# Autodesk Inventor assembly: Table
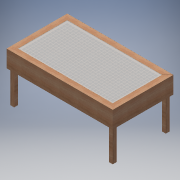
[picture p0: Inventor's stored thumbnail of the model, 180x180]
Saved by Autodesk Inventor 2016 (Build 200138000, 138)
## iProperties
Created: 2016-02-08
Part Number: Table
Document SubType Name: Assembly
Designer: ron
Author: ron
## Documents named in this file (16)
- C:\Users\ron\Desktop\Table\Table.iam
- C:\Users\ron\Desktop\Table\Parts\LedBoard.ipt
- C:\Users\ron\Desktop\Table\Parts\DividerWidth.ipt
- C:\Users\ron\Desktop\Table\Parts\DividerLength.ipt
- C:\Users\ron\Desktop\Table\Parts\Acrylitep95.ipt
- C:\Users\ron\Desktop\Table\Parts\LegStandard.ipt
- C:\Users\ron\Desktop\Table\Parts\Glass.ipt
- C:\Users\ron\Desktop\Table\Parts\LegOutlet.ipt
- C:\Users\ron\Desktop\Table\Parts\SideWidth.ipt
- C:\Users\ron\Desktop\Table\Parts\SideLength.ipt
- C:\Users\ron\Desktop\Table\Parts\SideWidthOutlet.ipt
- C:\Users\ron\Desktop\Table\Parts\SideLengthOutlet.ipt
- C:\Users\ron\Desktop\Table\Parts\SupportWedge.ipt
- C:\Users\ron\Desktop\Table\Parts\Bottom.ipt
- C:\Users\ron\Desktop\Table\Parts\PowerSupply.ipt
- C:\Users\ron\Desktop\Table\Parts\Magnet.ipt
## Components (72 placed, 15 different names)
1. LedBoard:1 — Flush:1, Flush:2, Flush:3, Flush:4, Flush:5, Flush:7, Flush:8, Flush:10, Flush:11, Flush:13, Flush:14, Flush:16, Flush:17, Flush:19, Flush:20, Flush:22, Flush:23, Flush:25, Flush:26, Flush:28, Flush:29, Flush:31, Flush:32, Flush:34, Flush:36, Flush:37, Flush:38, Flush:40, Flush:41, Flush:43, Flush:44, Flush:46, Flush:47, Flush:49, Flush:50, Flush:52, Flush:53, Flush:55, Flush:56, Flush:58, Flush:59, Flush:61, Flush:62, Flush:64, Flush:65, Flush:67, Flush:68, Flush:70, Flush:71, Flush:73, Flush:74, Flush:76, Flush:77, Flush:79, Flush:80, Flush:82, Flush:83, Flush:85, Flush:86, Flush:88, Flush:89, Flush:91, Flush:92, Flush:94, Flush:96, Mate:1, Flush:97, Flush:98, Mate:2, Flush:99, Mate:3, Flush:101, Mate:4, Flush:103, Mate:5, Flush:105, Mate:6, Flush:107, Flush:109, Mate:7, Mate:8, Flush:111, Mate:9, Flush:113, Mate:10, Flush:115, Mate:11, Flush:117, Mate:12, Flush:119, Mate:13, Flush:121, Mate:14, Flush:123, Mate:15, Flush:125, Flush:127, Flush:128, Mate:17, Mate:18, Mate:22, Mate:23, Mate:25, Mate:26, Mate:30, Mate:60, Mate:61, Mate:64, Mate:70, Mate:73, Mate:76, Mate:79
2. DividerWidth:1 — Flush:64, Flush:65, Flush:66, Flush:69
3. DividerWidth:2 — Flush:58, Flush:59, Flush:60, Flush:63
4. DividerWidth:3 — Flush:40, Flush:41, Flush:42, Flush:45
5. DividerWidth:4 — Flush:31, Flush:32, Flush:33, Flush:35
6. DividerWidth:5 — Flush:70, Flush:71, Flush:72, Flush:75
7. DividerWidth:6 — Flush:61, Flush:62, Flush:63, Flush:66
8. DividerWidth:7 — Flush:49, Flush:50, Flush:51, Flush:54
9. DividerWidth:8 — Flush:19, Flush:20, Flush:21, Flush:24
10. DividerWidth:9 — Flush:28, Flush:29, Flush:30, Flush:33
11. DividerWidth:10 — Flush:34, Flush:35, Flush:36, Flush:39, Mate:16
12. DividerWidth:11 — Flush:73, Flush:74, Flush:75, Flush:78
13. DividerWidth:12 — Flush:79, Flush:80, Flush:81, Flush:84
14. DividerWidth:13 — Flush:85, Flush:86, Flush:87, Flush:90
15. DividerWidth:14 — Flush:52, Flush:53, Flush:54, Flush:57
16. DividerWidth:15 — Flush:46, Flush:47, Flush:48, Flush:51
17. DividerWidth:16 — Flush:10, Flush:11, Flush:12, Flush:15
18. DividerWidth:17 — Flush:7, Flush:8, Flush:9, Flush:12
19. DividerWidth:18 — Flush:13, Flush:14, Flush:15, Flush:18, Flush:21
20. DividerWidth:19 — Flush:1, Flush:2, Flush:3, Flush:6
21. DividerWidth:20 — Flush:43, Flush:44, Flush:45, Flush:48
22. DividerWidth:21 — Flush:55, Flush:56, Flush:57, Flush:60
23. DividerWidth:22 — Flush:25, Flush:26, Flush:27, Flush:30
24. DividerWidth:23 — Flush:4, Flush:5, Flush:6, Flush:9
25. DividerWidth:24 — Flush:16, Flush:17, Flush:18
26. DividerWidth:25 — Flush:22, Flush:23, Flush:24, Flush:27
27. DividerWidth:26 — Flush:37, Flush:38, Flush:39, Flush:42
28. DividerWidth:27 — Flush:67, Flush:68, Flush:69, Flush:72
29. DividerWidth:28 — Flush:76, Flush:77, Flush:78, Flush:81
30. DividerWidth:29 — Flush:82, Flush:83, Flush:84, Flush:87
31. DividerWidth:30 — Flush:91, Flush:92, Flush:93, Flush:95
32. DividerWidth:31 — Flush:88, Flush:89, Flush:90, Flush:93
33. DividerLength:1 — Mate:5, Flush:105, Flush:106, Flush:108
34. DividerLength:2 — Mate:10, Flush:115, Flush:116, Flush:118
35. DividerLength:3 — Mate:1, Flush:97, Flush:98, Flush:100
36. DividerLength:4 — Mate:11, Flush:117, Flush:118, Flush:120
37. DividerLength:5 — Flush:109, Mate:7, Flush:110, Flush:112
38. DividerLength:6 — Mate:3, Flush:101, Flush:102, Flush:104
39. DividerLength:7 — Mate:13, Flush:121, Flush:122, Flush:124
40. DividerLength:8 — Mate:8, Flush:111, Flush:112, Flush:114
41. DividerLength:9 — Mate:4, Flush:103, Flush:104, Flush:106
42. DividerLength:10 — Mate:12, Flush:119, Flush:120, Flush:122
43. DividerLength:11 — Mate:15, Flush:125, Flush:126
44. DividerLength:12 — Mate:14, Flush:123, Flush:124, Flush:126
45. DividerLength:13 — Mate:9, Flush:113, Flush:114, Flush:116
46. DividerLength:14 — Mate:2, Flush:99, Flush:100, Flush:102
47. DividerLength:15 — Mate:6, Flush:107, Flush:108, Flush:110
48. DividerWidth:32 — Flush:94, Flush:95, Flush:96
49. Acrylitep95:1 — Flush:127, Mate:16, Flush:128, Mate:19, Mate:20, Flush:129, Flush:130, Mate:21, Mate:24, Mate:31, Mate:39, Mate:59, Mate:62, Mate:68
50. LegStandard:1 — Mate:21, Mate:22, Mate:23, Mate:89, Mate:90, Flush:136
51. LegStandard:2 — Mate:24, Mate:25, Mate:26, Mate:91, Mate:92, Flush:137
52. LegStandard:3 — Mate:17, Mate:18, Mate:19, Mate:85, Mate:86, Flush:134
53. Glass:1 — Mate:20, Flush:129, Flush:130, Mate:32, Mate:41, Mate:42, Mate:65
54. SideWidth:1 — Mate:30, Mate:31, Mate:32, Mate:42, Mate:66, Mate:69, Mate:77, Mate:80, Mate:97, Mate:98, Mate:99
55. SideLength:2 — Mate:39, Mate:41, Mate:63, Mate:66, Mate:75, Mate:78, Mate:84, Mate:93, Mate:94, Flush:138, Mate:100, Mate:101, Mate:102
56. LegOutlet:1 — Mate:59, Mate:60, Mate:61, Mate:87, Mate:88, Flush:135
57. SideWidthOutlet:1 — Mate:62, Mate:63, Mate:64, Mate:65, Mate:67, Mate:71, Mate:74, Flush:133, Mate:83, Mate:95, Flush:139, Mate:96
58. SideLengthOutlet:1 — Mate:67, Mate:68, Mate:69, Mate:72, Mate:81
59. SupportWedge:1 — Mate:76, Mate:77, Mate:78
60. SupportWedge:2 — Mate:73, Mate:74, Mate:75
61. SupportWedge:3 — Mate:79, Mate:80, Mate:81
62. SupportWedge:4 — Mate:70, Mate:71, Mate:72
63. Bottom:1 — Mate:82, Flush:131, Flush:132, Flush:133, Mate:83, Mate:84
64. PowerSupply:1 — Mate:82, Flush:131, Flush:132
65. Magnet:1 — Mate:93, Mate:94, Flush:138
66. Magnet:2 — Mate:95, Flush:139, Mate:96
67. Magnet:3 — Mate:85, Mate:86, Flush:134
68. Magnet:4 — Mate:89, Mate:90, Flush:136
69. Magnet:5 — Mate:87, Mate:88, Flush:135
70. Magnet:6 — Mate:91, Mate:92, Flush:137
71. Magnet:7 — Mate:97, Mate:98, Mate:99
72. Magnet:8 — Mate:100, Mate:101, Mate:102
## Relationships (215: Flush 139, Mate 76)
- Flush:1 (-50.8 mm): LedBoard:1 ↔ DividerWidth:19
- Flush:2: LedBoard:1 ↔ DividerWidth:19
- Flush:3 (34.925 mm): LedBoard:1 ↔ DividerWidth:19
- Flush:4: LedBoard:1 ↔ DividerWidth:23
- Flush:5 (-50.8 mm): LedBoard:1 ↔ DividerWidth:23
- Flush:6 (38.1 mm): DividerWidth:19 ↔ DividerWidth:23
- Flush:7 (-50.8 mm): LedBoard:1 ↔ DividerWidth:17
- Flush:8: LedBoard:1 ↔ DividerWidth:17
- Flush:9 (38.1 mm): DividerWidth:17 ↔ DividerWidth:23
- Flush:10 (-50.8 mm): LedBoard:1 ↔ DividerWidth:16
- Flush:11: LedBoard:1 ↔ DividerWidth:16
- Flush:12 (38.1 mm): DividerWidth:16 ↔ DividerWidth:17
- Flush:13 (-50.8 mm): LedBoard:1 ↔ DividerWidth:18
- Flush:14: LedBoard:1 ↔ DividerWidth:18
- Flush:15 (38.1 mm): DividerWidth:16 ↔ DividerWidth:18
- Flush:16 (-50.8 mm): LedBoard:1 ↔ DividerWidth:24
- Flush:17: LedBoard:1 ↔ DividerWidth:24
- Flush:18 (-38.1 mm): DividerWidth:18 ↔ DividerWidth:24
- Flush:19 (-50.8 mm): LedBoard:1 ↔ DividerWidth:8
- Flush:20: LedBoard:1 ↔ DividerWidth:8
- Flush:21 (38.1 mm): DividerWidth:8 ↔ DividerWidth:18
- Flush:22 (-50.8 mm): LedBoard:1 ↔ DividerWidth:25
- Flush:23: LedBoard:1 ↔ DividerWidth:25
- Flush:24 (38.1 mm): DividerWidth:8 ↔ DividerWidth:25
- Flush:25 (-50.8 mm): LedBoard:1 ↔ DividerWidth:22
- Flush:26: LedBoard:1 ↔ DividerWidth:22
- Flush:27 (38.1 mm): DividerWidth:22 ↔ DividerWidth:25
- Flush:28 (-50.8 mm): LedBoard:1 ↔ DividerWidth:9
- Flush:29: LedBoard:1 ↔ DividerWidth:9
- Flush:30 (38.1 mm): DividerWidth:9 ↔ DividerWidth:22
- Flush:31 (-50.8 mm): LedBoard:1 ↔ DividerWidth:4
- Flush:32: LedBoard:1 ↔ DividerWidth:4
- Flush:33 (38.1 mm): DividerWidth:4 ↔ DividerWidth:9
- Flush:34: LedBoard:1 ↔ DividerWidth:10
- Flush:35 (38.1 mm): DividerWidth:4 ↔ DividerWidth:10
- Flush:36 (-50.8 mm): LedBoard:1 ↔ DividerWidth:10
- Flush:37: LedBoard:1 ↔ DividerWidth:26
- Flush:38 (-50.8 mm): LedBoard:1 ↔ DividerWidth:26
- Flush:39 (38.1 mm): DividerWidth:10 ↔ DividerWidth:26
- Flush:40: LedBoard:1 ↔ DividerWidth:3
- Flush:41 (-50.8 mm): LedBoard:1 ↔ DividerWidth:3
- Flush:42 (38.1 mm): DividerWidth:3 ↔ DividerWidth:26
- Flush:43: LedBoard:1 ↔ DividerWidth:20
- Flush:44 (-50.8 mm): LedBoard:1 ↔ DividerWidth:20
- Flush:45 (38.1 mm): DividerWidth:3 ↔ DividerWidth:20
- Flush:46: LedBoard:1 ↔ DividerWidth:15
- Flush:47 (-50.8 mm): LedBoard:1 ↔ DividerWidth:15
- Flush:48 (38.1 mm): DividerWidth:15 ↔ DividerWidth:20
- Flush:49: LedBoard:1 ↔ DividerWidth:7
- Flush:50 (-50.8 mm): LedBoard:1 ↔ DividerWidth:7
- Flush:51 (38.1 mm): DividerWidth:7 ↔ DividerWidth:15
- Flush:52: LedBoard:1 ↔ DividerWidth:14
- Flush:53 (-50.8 mm): LedBoard:1 ↔ DividerWidth:14
- Flush:54 (38.1 mm): DividerWidth:7 ↔ DividerWidth:14
- Flush:55: LedBoard:1 ↔ DividerWidth:21
- Flush:56 (-50.8 mm): LedBoard:1 ↔ DividerWidth:21
- Flush:57 (38.1 mm): DividerWidth:14 ↔ DividerWidth:21
- Flush:58: LedBoard:1 ↔ DividerWidth:2
- Flush:59 (-50.8 mm): LedBoard:1 ↔ DividerWidth:2
- Flush:60 (38.1 mm): DividerWidth:2 ↔ DividerWidth:21
- Flush:61: LedBoard:1 ↔ DividerWidth:6
- Flush:62 (-50.8 mm): LedBoard:1 ↔ DividerWidth:6
- Flush:63 (38.1 mm): DividerWidth:2 ↔ DividerWidth:6
- Flush:64: LedBoard:1 ↔ DividerWidth:1
- Flush:65 (-50.8 mm): LedBoard:1 ↔ DividerWidth:1
- Flush:66 (38.1 mm): DividerWidth:1 ↔ DividerWidth:6
- Flush:67: LedBoard:1 ↔ DividerWidth:27
- Flush:68 (-50.8 mm): LedBoard:1 ↔ DividerWidth:27
- Flush:69 (38.1 mm): DividerWidth:1 ↔ DividerWidth:27
- Flush:70: LedBoard:1 ↔ DividerWidth:5
- Flush:71 (-50.8 mm): LedBoard:1 ↔ DividerWidth:5
- Flush:72 (38.1 mm): DividerWidth:5 ↔ DividerWidth:27
- Flush:73: LedBoard:1 ↔ DividerWidth:11
- Flush:74 (-50.8 mm): LedBoard:1 ↔ DividerWidth:11
- Flush:75 (38.1 mm): DividerWidth:5 ↔ DividerWidth:11
- Flush:76: LedBoard:1 ↔ DividerWidth:28
- Flush:77 (50.8 mm): LedBoard:1 ↔ DividerWidth:28
- Flush:78 (38.1 mm): DividerWidth:11 ↔ DividerWidth:28
- Flush:79: LedBoard:1 ↔ DividerWidth:12
- Flush:80 (-50.8 mm): LedBoard:1 ↔ DividerWidth:12
- Flush:81 (38.1 mm): DividerWidth:12 ↔ DividerWidth:28
- Flush:82: LedBoard:1 ↔ DividerWidth:29
- Flush:83 (-50.8 mm): LedBoard:1 ↔ DividerWidth:29
- Flush:84 (38.1 mm): DividerWidth:12 ↔ DividerWidth:29
- Flush:85: LedBoard:1 ↔ DividerWidth:13
- Flush:86 (-50.8 mm): LedBoard:1 ↔ DividerWidth:13
- Flush:87 (38.1 mm): DividerWidth:13 ↔ DividerWidth:29
- Flush:88: LedBoard:1 ↔ DividerWidth:31
- Flush:89 (-50.8 mm): LedBoard:1 ↔ DividerWidth:31
- Flush:90 (38.1 mm): DividerWidth:13 ↔ DividerWidth:31
- Flush:91: LedBoard:1 ↔ DividerWidth:30
- Flush:92 (50.8 mm): LedBoard:1 ↔ DividerWidth:30
- Flush:93 (38.1 mm): DividerWidth:30 ↔ DividerWidth:31
- Flush:94: LedBoard:1 ↔ DividerWidth:32
- Flush:95 (38.1 mm): DividerWidth:30 ↔ DividerWidth:32
- Flush:96 (-50.8 mm): LedBoard:1 ↔ DividerWidth:32
- Mate:1: LedBoard:1 ↔ DividerLength:3
- Flush:97: LedBoard:1 ↔ DividerLength:3
- Flush:98 (38.1 mm): LedBoard:1 ↔ DividerLength:3
- Mate:2: LedBoard:1 ↔ DividerLength:14
- Flush:99: LedBoard:1 ↔ DividerLength:14
- Flush:100 (-38.1 mm): DividerLength:3 ↔ DividerLength:14
- Mate:3: LedBoard:1 ↔ DividerLength:6
- Flush:101: LedBoard:1 ↔ DividerLength:6
- Flush:102 (38.1 mm): DividerLength:6 ↔ DividerLength:14
- Mate:4: LedBoard:1 ↔ DividerLength:9
- Flush:103: LedBoard:1 ↔ DividerLength:9
- Flush:104 (38.1 mm): DividerLength:6 ↔ DividerLength:9
- Mate:5: LedBoard:1 ↔ DividerLength:1
- Flush:105: LedBoard:1 ↔ DividerLength:1
- Flush:106 (38.1 mm): DividerLength:1 ↔ DividerLength:9
- Mate:6: LedBoard:1 ↔ DividerLength:15
- Flush:107: LedBoard:1 ↔ DividerLength:15
- Flush:108 (38.1 mm): DividerLength:1 ↔ DividerLength:15
- Flush:109: LedBoard:1 ↔ DividerLength:5
- Mate:7: LedBoard:1 ↔ DividerLength:5
- Flush:110 (38.1 mm): DividerLength:5 ↔ DividerLength:15
- Mate:8: LedBoard:1 ↔ DividerLength:8
- Flush:111: LedBoard:1 ↔ DividerLength:8
- Flush:112 (38.1 mm): DividerLength:5 ↔ DividerLength:8
- Mate:9: LedBoard:1 ↔ DividerLength:13
- Flush:113: LedBoard:1 ↔ DividerLength:13
- Flush:114 (38.1 mm): DividerLength:8 ↔ DividerLength:13
- Mate:10: LedBoard:1 ↔ DividerLength:2
- Flush:115: LedBoard:1 ↔ DividerLength:2
- Flush:116 (38.1 mm): DividerLength:2 ↔ DividerLength:13
- Mate:11: LedBoard:1 ↔ DividerLength:4
- Flush:117: LedBoard:1 ↔ DividerLength:4
- Flush:118 (38.1 mm): DividerLength:2 ↔ DividerLength:4
- Mate:12: LedBoard:1 ↔ DividerLength:10
- Flush:119: LedBoard:1 ↔ DividerLength:10
- Flush:120 (38.1 mm): DividerLength:4 ↔ DividerLength:10
- Mate:13: LedBoard:1 ↔ DividerLength:7
- Flush:121: LedBoard:1 ↔ DividerLength:7
- Flush:122 (38.1 mm): DividerLength:7 ↔ DividerLength:10
- Mate:14: LedBoard:1 ↔ DividerLength:12
- Flush:123: LedBoard:1 ↔ DividerLength:12
- Flush:124 (38.1 mm): DividerLength:7 ↔ DividerLength:12
- Mate:15: LedBoard:1 ↔ DividerLength:11
- Flush:125: LedBoard:1 ↔ DividerLength:11
- Flush:126 (38.1 mm): DividerLength:11 ↔ DividerLength:12
- Flush:127 (-25.4 mm): LedBoard:1 ↔ Acrylitep95:1
- Mate:16: DividerWidth:10 ↔ Acrylitep95:1
- Flush:128 (-25.4 mm): LedBoard:1 ↔ Acrylitep95:1
- Mate:17 (25.4 mm): LedBoard:1 ↔ LegStandard:3
- Mate:18 (25.4 mm): LedBoard:1 ↔ LegStandard:3
- Mate:19 (38.1 mm): Acrylitep95:1 ↔ LegStandard:3
- Mate:20: Acrylitep95:1 ↔ Glass:1
- Flush:129: Acrylitep95:1 ↔ Glass:1
- Flush:130: Acrylitep95:1 ↔ Glass:1
- Mate:21 (38.1 mm): Acrylitep95:1 ↔ LegStandard:1
- Mate:22 (25.4 mm): LedBoard:1 ↔ LegStandard:1
- Mate:23 (25.4 mm): LedBoard:1 ↔ LegStandard:1
- Mate:24 (38.1 mm): Acrylitep95:1 ↔ LegStandard:2
- Mate:25 (25.4 mm): LedBoard:1 ↔ LegStandard:2
- Mate:26 (25.4 mm): LedBoard:1 ↔ LegStandard:2
- Mate:30: LedBoard:1 ↔ SideWidth:1
- Mate:31: Acrylitep95:1 ↔ SideWidth:1
- Mate:32: Glass:1 ↔ SideWidth:1
- Mate:39: Acrylitep95:1 ↔ SideLength:2
- Mate:41: Glass:1 ↔ SideLength:2
- Mate:42: Glass:1 ↔ SideWidth:1
- Mate:59 (38.1 mm): Acrylitep95:1 ↔ LegOutlet:1
- Mate:60 (25.4 mm): LedBoard:1 ↔ LegOutlet:1
- Mate:61 (25.4 mm): LedBoard:1 ↔ LegOutlet:1
- Mate:62: Acrylitep95:1 ↔ SideWidthOutlet:1
- Mate:63: SideLength:2 ↔ SideWidthOutlet:1
- Mate:64: LedBoard:1 ↔ SideWidthOutlet:1
- Mate:65: Glass:1 ↔ SideWidthOutlet:1
- Mate:66: SideWidth:1 ↔ SideLength:2
- Mate:67: SideWidthOutlet:1 ↔ SideLengthOutlet:1
- Mate:68: Acrylitep95:1 ↔ SideLengthOutlet:1
- Mate:69: SideWidth:1 ↔ SideLengthOutlet:1
- Mate:70: LedBoard:1 ↔ SupportWedge:4
- Mate:71: SideWidthOutlet:1 ↔ SupportWedge:4
- Mate:72: SideLengthOutlet:1 ↔ SupportWedge:4
- Mate:73: LedBoard:1 ↔ SupportWedge:2
- Mate:74: SideWidthOutlet:1 ↔ SupportWedge:2
- Mate:75: SideLength:2 ↔ SupportWedge:2
- Mate:76: LedBoard:1 ↔ SupportWedge:1
- Mate:77: SideWidth:1 ↔ SupportWedge:1
- Mate:78: SideLength:2 ↔ SupportWedge:1
- Mate:79: LedBoard:1 ↔ SupportWedge:3
- Mate:80: SideWidth:1 ↔ SupportWedge:3
- Mate:81: SideLengthOutlet:1 ↔ SupportWedge:3
- Mate:82: Bottom:1 ↔ PowerSupply:1
- Flush:131 (50.8 mm): Bottom:1 ↔ PowerSupply:1
- Flush:132 (50.8 mm): Bottom:1 ↔ PowerSupply:1
- Flush:133: SideWidthOutlet:1 ↔ Bottom:1
- Mate:83: SideWidthOutlet:1 ↔ Bottom:1
- Mate:84: SideLength:2 ↔ Bottom:1
- Mate:85: LegStandard:3 ↔ Magnet:3
- Mate:86: LegStandard:3 ↔ Magnet:3
- Flush:134: LegStandard:3 ↔ Magnet:3
- Mate:87: LegOutlet:1 ↔ Magnet:5
- Mate:88: LegOutlet:1 ↔ Magnet:5
- Flush:135: LegOutlet:1 ↔ Magnet:5
- Mate:89: LegStandard:1 ↔ Magnet:4
- Mate:90: LegStandard:1 ↔ Magnet:4
- Flush:136: LegStandard:1 ↔ Magnet:4
- Mate:91: LegStandard:2 ↔ Magnet:6
- Mate:92: LegStandard:2 ↔ Magnet:6
- Flush:137: LegStandard:2 ↔ Magnet:6
- Mate:93: SideLength:2 ↔ Magnet:1
- Mate:94: SideLength:2 ↔ Magnet:1
- Flush:138: SideLength:2 ↔ Magnet:1
- Mate:95: SideWidthOutlet:1 ↔ Magnet:2
- Flush:139: SideWidthOutlet:1 ↔ Magnet:2
- Mate:96: SideWidthOutlet:1 ↔ Magnet:2
- Mate:97: SideWidth:1 ↔ Magnet:7
- Mate:98: SideWidth:1 ↔ Magnet:7
- Mate:99: SideWidth:1 ↔ Magnet:7
- Mate:100: SideLength:2 ↔ Magnet:8
- Mate:101: SideLength:2 ↔ Magnet:8
- Mate:102: SideLength:2 ↔ Magnet:8
